# Autodesk Inventor assembly: PC104_EM-113 Assembly
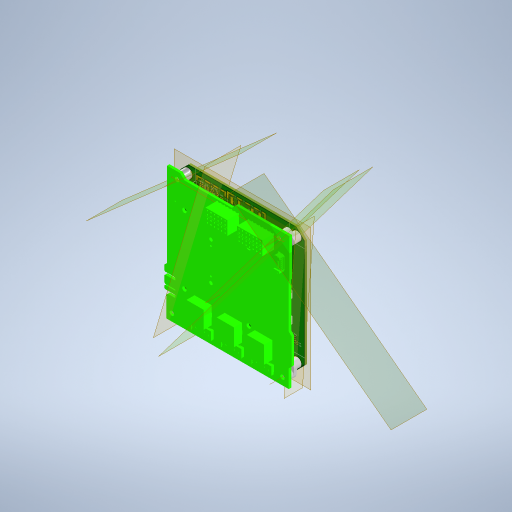
[picture p0: Inventor's stored thumbnail of the model, 512x512]
Saved by Autodesk Inventor 2024 (Build 280153000, 153)
## iProperties
Created: 2023-04-20
Part Number: PC104_EM-113 Assembly
Document SubType Name: Assembly
Designer: Owner
Author: Owner
## Documents named in this file (7)
- C:\Users\Owner\Desktop\AMSAT\Models\DAM parts\PC104_EM-113 Assembly.iam
- C:\Users\Owner\Desktop\AMSAT\Models\Frequent used files\CAD_backup_frequent_files_20200629 (1)\PCB_LT_ICR.iam
- C:\Users\Owner\Desktop\AMSAT\Models\ISISpace\ISISpace\isispace-icepsv2-e-1_typeb.ipt
- C:\Users\Owner\Desktop\AMSAT\Models\DAM parts\PC104_EM-113 standoff_4.563.ipt
- C:\Users\Owner\Desktop\AMSAT\Models\PC104_EM-113 standoff_4.746.ipt
- C:\Users\Owner\Desktop\AMSAT\Models\PC104_EM-113 standoff_3.57.ipt
- C:\Users\Owner\Desktop\AMSAT\Models\PC104_EM-113 standoff_3.268.ipt
## Components (6 placed, 6 different names)
1. PCB_LT_ICR:1 [sub-assembly] — Flush:1, Flush:2, Mate:1, Mate:2, Mate:5, Mate:7, Mate:8, Mate:11, Mate:12, Mate:13, Mate:15, Mate:18, Mate:24, Mate:27, Mate:28, Mate:29
2. isispace-icepsv2-e-1_typeb:1 — Flush:1, Flush:2, Mate:3, Mate:6, Mate:9, Mate:10, Mate:14, Mate:16, Mate:17, Mate:19, Mate:20
3. PC104_EM-113 standoff_4.563:1 — Mate:1, Mate:2, Angle:1
4. PC104_EM-113 standoff_4.746:1 — Angle:2, Mate:12, Mate:13, Mate:14
5. PC104_EM-113 standoff_3.57:1 — Mate:15, Mate:16, Mate:17
6. PC104_EM-113 standoff_3.268:1 — Mate:18, Angle:3
## Relationships (39: Mate 32, Angle 5, Flush 2)
- Flush:1 (-1.75 mm): PCB_LT_ICR:1 ↔ isispace-icepsv2-e-1_typeb:1
- Flush:2 (-0.75 mm): PCB_LT_ICR:1 ↔ isispace-icepsv2-e-1_typeb:1
- Mate:1: PCB_LT_ICR:1 ↔ PC104_EM-113 standoff_4.563:1
- Mate:2: PCB_LT_ICR:1 ↔ PC104_EM-113 standoff_4.563:1
- Mate:3: isispace-icepsv2-e-1_typeb:1
- Mate:4
- Mate:5: PCB_LT_ICR:1
- Angle:1 (180 deg): PC104_EM-113 standoff_4.563:1
- Mate:6: isispace-icepsv2-e-1_typeb:1
- Mate:7: PCB_LT_ICR:1
- Mate:8: PCB_LT_ICR:1
- Mate:9: isispace-icepsv2-e-1_typeb:1
- Mate:10: isispace-icepsv2-e-1_typeb:1
- Mate:11: PCB_LT_ICR:1
- Angle:2 (180 deg): PC104_EM-113 standoff_4.746:1
- Mate:12: PCB_LT_ICR:1 ↔ PC104_EM-113 standoff_4.746:1
- Mate:13: PCB_LT_ICR:1 ↔ PC104_EM-113 standoff_4.746:1
- Mate:14: isispace-icepsv2-e-1_typeb:1 ↔ PC104_EM-113 standoff_4.746:1
- Mate:15: PCB_LT_ICR:1 ↔ PC104_EM-113 standoff_3.57:1
- Mate:16: isispace-icepsv2-e-1_typeb:1 ↔ PC104_EM-113 standoff_3.57:1
- Mate:17: isispace-icepsv2-e-1_typeb:1 ↔ PC104_EM-113 standoff_3.57:1
- Mate:18: PCB_LT_ICR:1 ↔ PC104_EM-113 standoff_3.268:1
- Angle:3 (180 deg): PC104_EM-113 standoff_3.268:1
- Mate:19: isispace-icepsv2-e-1_typeb:1
- Mate:20: isispace-icepsv2-e-1_typeb:1
- Mate:21
- Mate:22
- Mate:23
- Mate:24: PCB_LT_ICR:1
- Mate:25
- Mate:26
- Angle:4 (90 deg)
- Mate:27: PCB_LT_ICR:1
- Angle:5 (90 deg)
- Mate:28: PCB_LT_ICR:1
- Mate:29: PCB_LT_ICR:1
- Mate:30
- Mate:31
- Mate:32
